# Autodesk Inventor assembly: Assembly1
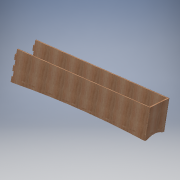
[picture p0: Inventor's stored thumbnail of the model, 180x180]
Saved by Autodesk Inventor 2016 (Build 200138000, 138)
## iProperties
Created: 2017-02-03
Part Number: Assembly1
Document SubType Name: Assembly
Designer: jwillauer
Author: jwillauer
## Documents named in this file (5)
- D:\New folder\87\Assembly1.iam
- D:\New folder\87\back.ipt
- D:\New folder\87\front.ipt
- D:\New folder\87\right side.ipt
- D:\New folder\87\bottom.ipt
## Components (4 placed, 4 different names)
1. back:1 — Flush:3, Flush:4, Flush:5, Flush:7
2. front:1 — Flush:1, Flush:2
3. right side:1 — Flush:1, Flush:2, Flush:3, Flush:4, Flush:5, Flush:6
4. bottom:1 — Flush:6, Flush:7
## Relationships (7: Flush 7)
- Flush:1: front:1 ↔ right side:1
- Flush:2: front:1 ↔ right side:1
- Flush:3: back:1 ↔ right side:1
- Flush:4: back:1 ↔ right side:1
- Flush:5: back:1 ↔ right side:1
- Flush:6: right side:1 ↔ bottom:1
- Flush:7: back:1 ↔ bottom:1
